# Autodesk Inventor assembly: !drivetrain
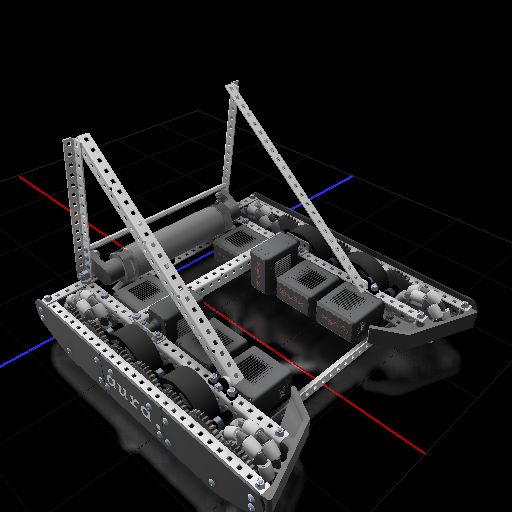
[picture p0: Inventor's stored thumbnail of the model, 512x512]
Saved by Autodesk Inventor 2025.2 (Build 292293000, 293)
## iProperties
Created: 2025-11-15
Part Number: !drivetrain
Document SubType Name: Assembly
Designer: cloudy
Author: cloudy
## Documents named in this file (53)
- C:\Users\cloudy\Documents\AURA_CAD\15\Drivetrain\!drivetrain.iam
- C:\Users\cloudy\Documents\AURA_CAD\15\Drivetrain\Wheels\Omni\2.75\2.75 Omni Assembly.iam
- C:\Users\cloudy\Documents\AURA_CAD\!lib\Structure\C Channel\Aluminum 1x2x1\Alu C 1x2x1x28.ipt
- C:\Users\cloudy\Documents\AURA_CAD\!lib\Structure\Hardware\Screw Steel - Star\SScrew Star Smooth 2.000.ipt
- C:\Users\cloudy\Documents\AURA_CAD\!lib\Structure\Hardware\Screw Steel - Star.ipt
- C:\Users\cloudy\Documents\AURA_CAD\!lib\Structure\Hardware\Nut Keps.ipt
- C:\Users\cloudy\Documents\AURA_CAD\!lib\Motion\Shaft LS\LS Pillow Bearing Block.ipt
- C:\Users\cloudy\Documents\AURA_CAD\!lib\Structure\C Channel\Aluminum 1x3x1 Half\Alu C Half 1x3x1x19.ipt
- C:\Users\cloudy\Documents\AURA_CAD\!lib\Structure\C Channel\Aluminum 1x2x1\Alu C 1x2x1x26.ipt
- C:\Users\cloudy\Documents\AURA_CAD\!lib\Structure\C Channel\Aluminum 1x3x1\Alu C 1x3x1x27.ipt
- C:\Users\cloudy\Documents\AURA_CAD\15\Drivetrain\Gears\26t_no_screwholes.ipt
- C:\Users\cloudy\Documents\AURA_CAD\!lib\Electronics\Motors with Screws\AluM-StarS.iam
- C:\Users\cloudy\Documents\AURA_CAD\!lib\Electronics\Motors with Screws.iam
- C:\Users\cloudy\Documents\AURA_CAD\15\Drivetrain\bearing_2 long.ipt
- C:\Users\cloudy\Documents\AURA_CAD\!lib\Motion\Spacers\Spacer Nylon .500 OD\NSpacer White .500 OD x .125.ipt
- C:\Users\cloudy\Documents\AURA_CAD\!lib\Motion\Spacers\Spacer Nylon .500 OD.ipt
- C:\Users\cloudy\Documents\AURA_CAD\!lib\Motion\Spacers\Spacer Nylon .375 OD\NSpacer .375 OD x .500.ipt
- C:\Users\cloudy\Documents\AURA_CAD\!lib\Motion\Spacers\Spacer Nylon .375 OD.ipt
- C:\Users\cloudy\Documents\AURA_CAD\!lib\Motion\Spacers\Spacer Nylon .375 OD\NSpacer .375 OD x .250.ipt
- C:\Users\cloudy\Documents\AURA_CAD\!lib\Motion\Shaft LS\Bearing Flat - Drilled.ipt
- C:\Users\cloudy\Documents\AURA_CAD\!lib\Motion\Shaft LS\Shaft Collar Metal\Shaft Collar No Screw.iam
- C:\Users\cloudy\Documents\AURA_CAD\!lib\Motion\Shaft LS\Shaft Collar Metal.iam
- C:\Users\cloudy\Documents\AURA_CAD\!lib\Structure\Standoff\Standoff 3.00.ipt
- C:\Users\cloudy\Documents\AURA_CAD\!lib\Structure\Standoff.ipt
- C:\Users\cloudy\Documents\AURA_CAD\!lib\Motion\Spacers\Spacer Nylon .375 OD\NSpacer .375 OD x .375.ipt
- C:\Users\cloudy\Documents\AURA_CAD\!lib\Motion\Spacers\Washer Steel\SWasher .375 OD x .062500.ipt
- C:\Users\cloudy\Documents\AURA_CAD\!lib\Motion\Spacers\Washer Steel.ipt
- C:\Users\cloudy\Documents\AURA_CAD\!lib\Structure\C Channel\Aluminum 1x3x1 Half\Alu C Half 1x3x1x3.ipt
- C:\Users\cloudy\Documents\AURA_CAD\!lib\Structure\C Channel\Aluminum 1x3x1 Half\Alu C Half 1x3x1x23.ipt
- C:\Users\cloudy\Documents\AURA_CAD\!lib\Structure\C Channel\Aluminum 1x3x1 Half\Alu C Half 1x3x1x15.ipt
- C:\Users\cloudy\Documents\AURA_CAD\!lib\Motion\Pneumatics\Legacy - SMC Pneumatics\Reservoir.ipt
- C:\Users\cloudy\Documents\AURA_CAD\15\cut_halfc.ipt
- C:\Users\cloudy\Documents\AURA_CAD\15\Drivetrain\Wheels\Traction\traction.iam
- C:\Users\cloudy\Documents\AURA_CAD\!lib\Structure\Hardware\Nut Nylock.ipt
- C:\Users\cloudy\Documents\AURA_CAD\15\ziptie.ipt
- C:\Users\cloudy\Documents\AURA_CAD\!lib\Motion\Shaft LS\Shaft LS Capped\Shaft LS Capped 3.0.ipt
- C:\Users\cloudy\Documents\AURA_CAD\!lib\Motion\Shaft LS\Shaft LS Capped.ipt
- C:\Users\cloudy\Documents\AURA_CAD\!lib\Structure\Hardware\Screw Steel - Star\SScrew Star Smooth .625.ipt
- C:\Users\cloudy\Documents\AURA_CAD\!lib\Structure\Hardware\Screw Steel - Star\SScrew Star Smooth .750.ipt
- C:\Users\cloudy\Documents\AURA_CAD\!lib\Structure\Hardware\Screw Steel - Star\SScrew Star Smooth .375.ipt
- C:\Users\cloudy\Documents\AURA_CAD\!lib\Structure\Hardware\Screw Steel - Star\SScrew Star Threaded 1.750.ipt
- C:\Users\cloudy\Documents\AURA_CAD\!lib\Structure\Hardware\Screw Steel - Star\SScrew Star Threaded .500.ipt
- C:\Users\cloudy\Documents\AURA_CAD\!lib\Structure\Standoff\Standoff 4.00.ipt
- C:\Users\cloudy\Documents\AURA_CAD\!lib\Structure\Standoff\Standoff .50.ipt
- C:\Users\cloudy\Documents\AURA_CAD\15\thing.ipt
- C:\Users\cloudy\Documents\AURA_CAD\15\thing_MIR.ipt
- C:\Users\cloudy\Documents\AURA_CAD\15\Drivetrain\funnel.ipt
- C:\Users\cloudy\Documents\AURA_CAD\!lib\Structure\C Channel\Aluminum 1x3x1 Half Thick Cut\Alu C Half Thick 1x3x1x20.ipt
- C:\Users\cloudy\Documents\AURA_CAD\!lib\Motion\Spacers\Spacer Nylon .375 OD\NSpacer .375 OD x .125.ipt
- C:\Users\cloudy\Documents\AURA_CAD\15\funnelFront.ipt
- C:\Users\cloudy\Documents\AURA_CAD\15\plate.ipt
- C:\Users\cloudy\Documents\AURA_CAD\!lib\Structure\Hardware\Screw Steel - Star\SScrew Star Smooth 1.250.ipt
- C:\Users\cloudy\Documents\AURA_CAD\!lib\Miscellaneous\iw_metal_02.bmp
## Components (277 placed, 43 different names)
1. Alu C 1x2x1x26:1 — Insert:10, Insert:19, Insert:20, Insert:26, Insert:36, Insert:40, Mate:22, Mate:23, Insert:41, Insert:42, Insert:43, Insert:47, Mate:24, Insert:51, Insert:67, Insert:90, Mate:37, Mate:38, Insert:102, Mate:44, Insert:110, Insert:117, Insert:122, Insert:123, Insert:126, Insert:144, Insert:154, Insert:157, Insert:163, Insert:164, Insert:165, Insert:170, Insert:171, Mate:92, Insert:313, Insert:315
2. SScrew Star Smooth 2.000:1 — Insert:10, Mate:26
3. 2.75 Omni Assembly:5 [sub-assembly] — Insert:46
4. SScrew Star Smooth 2.000:2 — Insert:20
5. SScrew Star Smooth 2.000:3 — Insert:19
6. 2.75 Omni Assembly:7 [sub-assembly] — Insert:44
7. Alu C Half 1x3x1x19:1 — Insert:26, Insert:161, Insert:162, Insert:264, Insert:265
8. Alu C 1x3x1x27:1 — Mate:15, Mate:16, Insert:32, Mate:34, Insert:72, Insert:108, Insert:126, Insert:141, Insert:150, Insert:155, Insert:156, Insert:158, Insert:167, Insert:168, Insert:169, Insert:257, Insert:258, Insert:260, Insert:262
9. 26t_no_screwholes:1 — Insert:52, Insert:56
10. 26t_no_screwholes:2 — Insert:53, Insert:55
11. 26t_no_screwholes:3 — Insert:54, Insert:57
12. Alu C 1x2x1x28:3 — Insert:32, Mate:26, Insert:52, Insert:53, Insert:54, Insert:58, Insert:59, Insert:60, Mate:27, Mate:28, Mate:29, Insert:61, Mate:30, Insert:62, Insert:63, Insert:64, Mate:31, Mate:32, Mate:33, Insert:124, Insert:125, Insert:127, Insert:128, Insert:129, Insert:130, Insert:131, Insert:132, Insert:133, Insert:134, Mate:49, Mate:50, Mate:51, Mate:52, Mate:53, Mate:54, Mate:55, Mate:56, Mate:57, Mate:58, Insert:135, Insert:136, Insert:137, Insert:138, Insert:152, Insert:283, Insert:284, Mate:93, Insert:294, Mate:95, Insert:297, Mate:97, Insert:314, Insert:316
13. AluM-StarS:1 [sub-assembly] — Insert:36, Mate:22
14. AluM-StarS:2 [sub-assembly] — Insert:40, Mate:23
15. AluM-StarS:3 [sub-assembly] — Insert:47, Mate:24
16. Nut Keps:1 — Insert:41, Insert:44
17. Nut Keps:2 — Insert:42, Insert:111
18. Nut Keps:3 — Insert:43, Insert:46
19. NSpacer White .500 OD x .125:2 — Insert:51
20. NSpacer .375 OD x .250:2 — Insert:56
21. NSpacer .375 OD x .250:3 — Insert:55
22. NSpacer .375 OD x .250:4 — Insert:57
23. bearing_2 long:3 — Insert:59, Mate:28
24. bearing_2 long:4 — Insert:61, Mate:30, Insert:112
25. bearing_2 long:5 — Insert:58, Mate:29
26. bearing_2 long:6 — Insert:60, Mate:27
27. Bearing Flat - Drilled:1 — Insert:62, Mate:33
28. Bearing Flat - Drilled:2 — Insert:64, Mate:31
29. Bearing Flat - Drilled:3 — Insert:63, Mate:32
30. Shaft Collar No Screw:1 [sub-assembly] — Insert:67, Mate:35, Insert:69, Insert:166
31. Shaft Collar No Screw:2 [sub-assembly] — Mate:34, Mate:35, Insert:68, Insert:74
32. Standoff 3.00:1 — Insert:70
33. NSpacer .375 OD x .500:5 — Insert:68
34. NSpacer .375 OD x .375:6 — Insert:69, Insert:70
35. NSpacer .375 OD x .500:7 — Insert:71, Insert:73
36. NSpacer .375 OD x .500:8 — Insert:71, Insert:72
37. SWasher .375 OD x .062500:1 — Insert:73
38. SWasher .375 OD x .062500:2 — Insert:74
39. Alu C Half 1x3x1x3:1 — Insert:90, Mate:37, Insert:91, Insert:147, Insert:148
40. AluM-StarS:7 [sub-assembly] — Insert:91, Mate:38
41. Alu C Half 1x3x1x23:1 — Mate:48, Insert:139, Insert:142
42. LS Pillow Bearing Block:2 — Insert:102, Mate:44, Insert:143, Insert:145, Insert:146
43. Shaft Collar No Screw:5 [sub-assembly] — Insert:108, Insert:109, Insert:159
44. Alu C Half 1x3x1x15:1 — Insert:109, Mate:48, Insert:160, Insert:270, Insert:279, Mate:90, Insert:280, Insert:281
45. Reservoir:1 — Mate:87, Mate:89
46. cut_halfc:1 — Insert:110, Insert:140, Insert:149, Mate:85
47. traction:1 [sub-assembly] — Insert:113
48. traction:2 [sub-assembly] — Insert:111, Insert:114
49. NSpacer .375 OD x .250:9 — Insert:112, Insert:113
50. Nut Nylock:1 — Insert:114
51. NSpacer .375 OD x .500:10 — Insert:116, Insert:117
52. NSpacer .375 OD x .375:11 — Insert:115
53. Shaft Collar No Screw:6 [sub-assembly] — Insert:115, Insert:116
54. NSpacer .375 OD x .500:12 — Insert:122
55. NSpacer .375 OD x .375:13
56. Shaft Collar No Screw:7 [sub-assembly]
57. NSpacer .375 OD x .500:14 — Insert:123
58. NSpacer .375 OD x .375:15
59. Shaft Collar No Screw:8 [sub-assembly]
60. ziptie:1 — Insert:125, Mate:56
61. ziptie:2 — Insert:127, Mate:57
62. ziptie:3 — Insert:128, Mate:55
63. ziptie:4 — Insert:124, Mate:58
64. ziptie:5 — Insert:129, Mate:53
65. ziptie:6 — Insert:130, Mate:54
66. ziptie:7 — Insert:131, Mate:52
67. ziptie:8 — Insert:133, Mate:50
68. ziptie:9 — Insert:132, Mate:51
69. ziptie:10 — Insert:134, Mate:49
70. Shaft LS Capped 3.0:1 — Insert:135
71. Shaft LS Capped 3.0:2 — Insert:136
72. Shaft LS Capped 3.0:3 — Insert:137
73. Shaft LS Capped 3.0:4 — Insert:138
74. NSpacer White .500 OD x .125:3 — Insert:139
75. NSpacer White .500 OD x .125:4 — Insert:140
76. NSpacer White .500 OD x .125:5 — Insert:141
77. SScrew Star Smooth .625:4 — Insert:142
78. Nut Nylock:2 — Insert:143
79. Nut Keps:4 — Insert:144
80. Nut Nylock:3 — Insert:146
81. Nut Nylock:4 — Insert:145
82. Nut Keps:5 — Insert:147
83. Nut Keps:6 — Insert:148
84. Nut Keps:7 — Insert:149
85. Nut Nylock:5 — Insert:150
86. NSpacer .375 OD x .500:16 — Insert:151, Insert:152
87. NSpacer .375 OD x .375:17 — Insert:151
88. NSpacer .375 OD x .500:18 — Insert:154
89. NSpacer .375 OD x .375:19
90. NSpacer .375 OD x .375:20 — Insert:155
91. NSpacer .375 OD x .375:21 — Insert:156
92. Nut Keps:8 — Insert:157
93. Nut Keps:9 — Insert:158
94. Nut Keps:10 — Insert:159
95. SScrew Star Smooth .625:5 — Insert:160
96. NSpacer .375 OD x .500:22 — Insert:161
97. SScrew Star Smooth .750:6 — Insert:162
98. SScrew Star Threaded .500:7 — Insert:164
99. SScrew Star Smooth .375:8 — Insert:163
100. SScrew Star Smooth .375:10 — Insert:165
101. SScrew Star Threaded .500:11 — Insert:166
102. SScrew Star Threaded 1.750:12 — Insert:167
103. SScrew Star Threaded 1.750:13 — Insert:168
104. SScrew Star Threaded 1.750:14 — Insert:169
105. SScrew Star Threaded .500:15 — Insert:170
106. SScrew Star Threaded .500:16 — Insert:171
107. Alu C 1x2x1x26:2 — Insert:172, Insert:173, Insert:174, Mate:60, Insert:178, Mate:61, Insert:179, Mate:62, Insert:180, Insert:182, Insert:183, Insert:185, Insert:186, Insert:197, Mate:71, Insert:204, Mate:72, Mate:73, Insert:206, Insert:213, Insert:216, Insert:219, Insert:239, Insert:246, Insert:248, Insert:252, Insert:253, Insert:255, Insert:256, Insert:258, Insert:263, Mate:91, Insert:317, Insert:319
108. SScrew Star Smooth 2.000:17 — Insert:172, Mate:59
109. 2.75 Omni Assembly:8 [sub-assembly] — Insert:184
110. SScrew Star Smooth 2.000:18 — Insert:173
111. SScrew Star Smooth 2.000:19 — Insert:174
112. 2.75 Omni Assembly:9 [sub-assembly] — Insert:181
113. 26t_no_screwholes:4 — Insert:177, Insert:187
114. 26t_no_screwholes:5 — Insert:176, Insert:188
115. 26t_no_screwholes:6 — Insert:175, Insert:189
116. Alu C 1x2x1x28:4 — Insert:175, Insert:176, Insert:177, Mate:59, Mate:63, Insert:190, Mate:64, Insert:191, Mate:65, Insert:192, Mate:66, Insert:193, Mate:67, Insert:194, Mate:68, Insert:195, Mate:69, Insert:196, Mate:75, Insert:222, Mate:76, Insert:223, Mate:77, Insert:224, Mate:78, Insert:225, Mate:79, Insert:226, Mate:80, Insert:227, Mate:81, Insert:228, Mate:82, Insert:229, Mate:83, Insert:230, Mate:84, Insert:231, Insert:232, Insert:233, Insert:234, Insert:235, Insert:244, Insert:257, Insert:282, Insert:285, Mate:94, Insert:295, Insert:296, Mate:96, Mate:98, Insert:318, Insert:320
117. AluM-StarS:8 [sub-assembly] — Mate:60, Insert:178
118. AluM-StarS:9 [sub-assembly] — Mate:61, Insert:179
119. AluM-StarS:10 [sub-assembly] — Mate:62, Insert:180
120. Nut Keps:11 — Insert:181, Insert:182
121. Nut Keps:12 — Insert:183, Insert:209
122. Nut Keps:13 — Insert:184, Insert:185
123. NSpacer White .500 OD x .125:6 — Insert:186
124. NSpacer .375 OD x .250:23 — Insert:187
125. NSpacer .375 OD x .250:24 — Insert:188
126. NSpacer .375 OD x .250:25 — Insert:189
127. bearing_2 long:7 — Mate:63, Insert:190
128. bearing_2 long:8 — Mate:64, Insert:191, Insert:211
129. bearing_2 long:9 — Mate:65, Insert:192
130. bearing_2 long:10 — Mate:66, Insert:193
131. Bearing Flat - Drilled:4 — Mate:67, Insert:194
132. Bearing Flat - Drilled:5 — Mate:68, Insert:195
133. Bearing Flat - Drilled:6 — Mate:69, Insert:196
134. Shaft Collar No Screw:9 [sub-assembly] — Insert:197, Mate:70, Insert:200, Insert:266
135. Shaft Collar No Screw:10 [sub-assembly] — Mate:70, Insert:198, Insert:203, Insert:261
136. Standoff 3.00:2 — Insert:199
137. NSpacer .375 OD x .500:26 — Insert:198
138. NSpacer .375 OD x .375:27 — Insert:199, Insert:200
139. NSpacer .375 OD x .500:28 — Insert:201, Insert:202
140. NSpacer .375 OD x .500:29 — Insert:201, Insert:262
141. SWasher .375 OD x .062500:3 — Insert:202, Insert:261
142. SWasher .375 OD x .062500:4 — Insert:203
143. Alu C Half 1x3x1x3:2 — Mate:71, Insert:204, Insert:205, Insert:242, Insert:243
144. AluM-StarS:11 [sub-assembly] — Mate:72, Insert:205
145. Alu C Half 1x3x1x23:2 — Insert:207, Mate:74, Insert:236, Insert:237
146. LS Pillow Bearing Block:3 — Mate:73, Insert:206, Insert:207, Insert:238, Insert:240, Insert:241
147. Shaft Collar No Screw:11 [sub-assembly] — Insert:208, Insert:249, Insert:259
148. Alu C Half 1x3x1x15:2 — Mate:74, Insert:208, Insert:250, Insert:269, Insert:271, Insert:272, Mate:88, Insert:273, Insert:274
149. traction:3 [sub-assembly] — Insert:210
150. traction:4 [sub-assembly] — Insert:209, Insert:212
151. NSpacer .375 OD x .250:30 — Insert:210, Insert:211
152. Nut Nylock:6 — Insert:212
153. NSpacer .375 OD x .500:31 — Insert:213, Insert:214
154. NSpacer .375 OD x .375:32 — Insert:215
155. Shaft Collar No Screw:12 [sub-assembly] — Insert:214, Insert:215
156. NSpacer .375 OD x .500:33 — Insert:216, Insert:217
157. NSpacer .375 OD x .375:34 — Insert:218
158. Shaft Collar No Screw:13 [sub-assembly] — Insert:217, Insert:218
159. NSpacer .375 OD x .500:35 — Insert:219, Insert:220
160. NSpacer .375 OD x .375:36 — Insert:221
161. Shaft Collar No Screw:14 [sub-assembly] — Insert:220, Insert:221
162. ziptie:11 — Mate:75, Insert:222
163. ziptie:12 — Mate:76, Insert:223
164. ziptie:13 — Mate:77, Insert:224
165. ziptie:14 — Mate:78, Insert:225
166. ziptie:15 — Mate:79, Insert:226
167. ziptie:16 — Mate:80, Insert:227
168. ziptie:17 — Mate:81, Insert:228
169. ziptie:18 — Mate:82, Insert:229
170. ziptie:19 — Mate:83, Insert:230
171. ziptie:20 — Mate:84, Insert:231
172. Shaft LS Capped 3.0:5 — Insert:232
173. Shaft LS Capped 3.0:6 — Insert:233
174. Shaft LS Capped 3.0:7 — Insert:234
175. Shaft LS Capped 3.0:8 — Insert:235
176. NSpacer White .500 OD x .125:7 — Insert:236
177. NSpacer White .500 OD x .125:8 — Mate:85
178. NSpacer White .500 OD x .125:9 — Insert:259, Insert:260
179. SScrew Star Smooth .625:20 — Insert:237
180. Nut Nylock:7 — Insert:238
181. Nut Keps:14 — Insert:239, Mate:86
182. Nut Nylock:8 — Insert:240
183. Nut Nylock:9 — Insert:241
184. Nut Keps:15 — Insert:242
185. Nut Keps:16 — Insert:243
186. Nut Keps:17
187. Nut Nylock:10
188. NSpacer .375 OD x .500:37 — Insert:244, Insert:245
189. NSpacer .375 OD x .375:38 — Insert:245
190. NSpacer .375 OD x .500:39 — Insert:246, Insert:247
191. NSpacer .375 OD x .375:40 — Insert:247
192. NSpacer .375 OD x .375:41
193. NSpacer .375 OD x .375:42
194. Nut Keps:18 — Insert:248
195. Nut Keps:19
196. Nut Keps:20 — Insert:249
197. SScrew Star Smooth .625:21 — Insert:250
198. NSpacer .375 OD x .500:43 — Insert:265, Mate:86
199. SScrew Star Smooth .750:22 — Insert:264
200. SScrew Star Smooth .375:24 — Insert:252
201. SScrew Star Smooth .375:25 — Insert:253
202. SScrew Star Threaded 1.750:27
203. SScrew Star Threaded 1.750:28
204. SScrew Star Threaded 1.750:29
205. SScrew Star Threaded .500:30 — Insert:255
206. SScrew Star Threaded .500:31 — Insert:256
207. SScrew Star Threaded .500:32 — Insert:263
208. SScrew Star Threaded .500:33 — Insert:266
209. Standoff 4.00:3 — Insert:267
210. Standoff 4.00:4 — Insert:268, Insert:269
211. Standoff .50:5 — Insert:267, Insert:268
212. SScrew Star Smooth .625:34 — Insert:271
213. SScrew Star Smooth .625:35 — Insert:270
214. thing:1 — Insert:272, Mate:88, Mate:89, Insert:275, Insert:276
215. SScrew Star Smooth .625:36 — Insert:274
216. SScrew Star Smooth .625:37 — Insert:273
217. Nut Nylock:11 — Insert:275
218. Nut Nylock:13 — Insert:276
219. thing_MIR:1 — Insert:277, Insert:278, Insert:279, Mate:90
220. SScrew Star Smooth .625:38 — Insert:281
221. SScrew Star Smooth .625:39 — Insert:280
222. Nut Nylock:14 — Insert:277
223. Nut Nylock:15 — Insert:278
224. funnel:2 — Insert:282, Mate:91
225. funnel:3 — Insert:283, Mate:92
226. Alu C Half Thick 1x3x1x20:1 — Insert:284, Mate:93, Insert:287, Insert:289, Flush:1
227. Alu C Half Thick 1x3x1x20:2 — Insert:285, Mate:94, Insert:291, Insert:293, Insert:298
228. NSpacer .375 OD x .500:44 — Insert:286, Insert:287
229. NSpacer .375 OD x .125:45 — Insert:286
230. NSpacer .375 OD x .500:46 — Insert:289
231. NSpacer .375 OD x .125:47
232. NSpacer .375 OD x .500:48 — Insert:291
233. NSpacer .375 OD x .125:49
234. NSpacer .375 OD x .500:50 — Insert:293
235. NSpacer .375 OD x .125:51
236. funnelFront:1 — Insert:295, Insert:321, Insert:322, Insert:323, Insert:324, Insert:325
237. funnelFront:2 — Insert:294, Mate:95, Insert:299, Insert:300, Insert:301, Insert:302, Insert:303
238. funnelFront:3 — Insert:296, Mate:96, Insert:330, Insert:331, Insert:332, Insert:333, Insert:334
239. funnelFront:4 — Insert:297, Mate:97, Insert:308, Insert:309, Insert:310, Insert:311, Insert:312
240. plate:1 — Flush:1, Insert:304, Insert:305, Insert:306, Insert:307
241. plate:2 — Insert:298, Mate:98, Insert:326, Insert:327, Insert:328, Insert:329
242. SScrew Star Smooth .375:40 — Insert:301
243. SScrew Star Smooth .375:41 — Insert:302
244. SScrew Star Smooth .375:42 — Insert:300
245. SScrew Star Smooth .375:43 — Insert:303
246. SScrew Star Smooth .375:44 — Insert:299
247. SScrew Star Smooth .375:45 — Insert:310
248. SScrew Star Smooth .375:46 — Insert:311
249. SScrew Star Smooth .375:47 — Insert:309
250. SScrew Star Smooth .375:48 — Insert:312
251. SScrew Star Smooth .375:49 — Insert:307
252. SScrew Star Smooth .375:50 — Insert:308
253. SScrew Star Smooth .375:51 — Insert:306
254. SScrew Star Smooth .375:52 — Insert:304
255. SScrew Star Smooth .375:53 — Insert:305
256. Nut Nylock:16 — Insert:315
257. SScrew Star Smooth 1.250:54 — Insert:314
258. Nut Nylock:17 — Insert:316
259. SScrew Star Smooth 1.250:55 — Insert:313
260. Nut Nylock:18 — Insert:319
261. SScrew Star Smooth 1.250:56 — Insert:318
262. Nut Nylock:19 — Insert:320
263. SScrew Star Smooth 1.250:57 — Insert:317
264. SScrew Star Smooth .375:58 — Insert:321
265. SScrew Star Smooth .375:59 — Insert:325
266. SScrew Star Smooth .375:60 — Insert:322
267. SScrew Star Smooth .375:61 — Insert:324
268. SScrew Star Smooth .375:62 — Insert:323
269. SScrew Star Smooth .375:63 — Insert:333
270. SScrew Star Smooth .375:64 — Insert:329
271. SScrew Star Smooth .375:65 — Insert:330
272. SScrew Star Smooth .375:66 — Insert:328
273. SScrew Star Smooth .375:67 — Insert:334
274. SScrew Star Smooth .375:68 — Insert:332
275. SScrew Star Smooth .375:69 — Insert:331
276. SScrew Star Smooth .375:70 — Insert:326
277. SScrew Star Smooth .375:71 — Insert:327
## Relationships (334: Insert 264, Mate 69, Flush 1)
- Insert:10: Alu C 1x2x1x26:1 ↔ SScrew Star Smooth 2.000:1
- Insert:19: Alu C 1x2x1x26:1 ↔ SScrew Star Smooth 2.000:3
- Insert:20: Alu C 1x2x1x26:1 ↔ SScrew Star Smooth 2.000:2
- Insert:26 (12.7 mm): Alu C 1x2x1x26:1 ↔ Alu C Half 1x3x1x19:1
- Mate:15: Alu C 1x3x1x27:1
- Mate:16: Alu C 1x3x1x27:1
- Insert:32: Alu C 1x3x1x27:1 ↔ Alu C 1x2x1x28:3
- Insert:36: Alu C 1x2x1x26:1 ↔ AluM-StarS:1
- Insert:40: Alu C 1x2x1x26:1 ↔ AluM-StarS:2
- Mate:22: Alu C 1x2x1x26:1 ↔ AluM-StarS:1
- Mate:23: Alu C 1x2x1x26:1 ↔ AluM-StarS:2
- Insert:41: Alu C 1x2x1x26:1 ↔ Nut Keps:1
- Insert:42: Alu C 1x2x1x26:1 ↔ Nut Keps:2
- Insert:43: Alu C 1x2x1x26:1 ↔ Nut Keps:3
- Insert:44 (0.7937 mm): 2.75 Omni Assembly:7 ↔ Nut Keps:1
- Insert:46 (0.7937 mm): 2.75 Omni Assembly:5 ↔ Nut Keps:3
- Insert:47: Alu C 1x2x1x26:1 ↔ AluM-StarS:3
- Mate:24: Alu C 1x2x1x26:1 ↔ AluM-StarS:3
- Insert:51: Alu C 1x2x1x26:1 ↔ NSpacer White .500 OD x .125:2
- Mate:26: SScrew Star Smooth 2.000:1 ↔ Alu C 1x2x1x28:3
- Insert:52 (13.4938 mm): 26t_no_screwholes:1 ↔ Alu C 1x2x1x28:3
- Insert:53 (13.4938 mm): 26t_no_screwholes:2 ↔ Alu C 1x2x1x28:3
- Insert:54 (13.4938 mm): 26t_no_screwholes:3 ↔ Alu C 1x2x1x28:3
- Insert:55: 26t_no_screwholes:2 ↔ NSpacer .375 OD x .250:3
- Insert:56: 26t_no_screwholes:1 ↔ NSpacer .375 OD x .250:2
- Insert:57: 26t_no_screwholes:3 ↔ NSpacer .375 OD x .250:4
- Insert:58: Alu C 1x2x1x28:3 ↔ bearing_2 long:5
- Insert:59: Alu C 1x2x1x28:3 ↔ bearing_2 long:3
- Insert:60: Alu C 1x2x1x28:3 ↔ bearing_2 long:6
- Mate:27: Alu C 1x2x1x28:3 ↔ bearing_2 long:6
- Mate:28: Alu C 1x2x1x28:3 ↔ bearing_2 long:3
- Mate:29: Alu C 1x2x1x28:3 ↔ bearing_2 long:5
- Insert:61: Alu C 1x2x1x28:3 ↔ bearing_2 long:4
- Mate:30: Alu C 1x2x1x28:3 ↔ bearing_2 long:4
- Insert:62: Alu C 1x2x1x28:3 ↔ Bearing Flat - Drilled:1
- Insert:63: Alu C 1x2x1x28:3 ↔ Bearing Flat - Drilled:3
- Insert:64: Alu C 1x2x1x28:3 ↔ Bearing Flat - Drilled:2
- Mate:31: Alu C 1x2x1x28:3 ↔ Bearing Flat - Drilled:2
- Mate:32: Alu C 1x2x1x28:3 ↔ Bearing Flat - Drilled:3
- Mate:33: Alu C 1x2x1x28:3 ↔ Bearing Flat - Drilled:1
- Insert:67: Alu C 1x2x1x26:1 ↔ Shaft Collar No Screw:1
- Mate:34: Alu C 1x3x1x27:1 ↔ Shaft Collar No Screw:2
- Mate:35: Shaft Collar No Screw:1 ↔ Shaft Collar No Screw:2
- Insert:68: Shaft Collar No Screw:2 ↔ NSpacer .375 OD x .500:5
- Insert:69: Shaft Collar No Screw:1 ↔ NSpacer .375 OD x .375:6
- Insert:70: Standoff 3.00:1 ↔ NSpacer .375 OD x .375:6
- Insert:71: NSpacer .375 OD x .500:7 ↔ NSpacer .375 OD x .500:8
- Insert:72: Alu C 1x3x1x27:1 ↔ NSpacer .375 OD x .500:8
- Insert:73: NSpacer .375 OD x .500:7 ↔ SWasher .375 OD x .062500:1
- Insert:74: Shaft Collar No Screw:2 ↔ SWasher .375 OD x .062500:2
- Insert:90: Alu C 1x2x1x26:1 ↔ Alu C Half 1x3x1x3:1
- Mate:37: Alu C 1x2x1x26:1 ↔ Alu C Half 1x3x1x3:1
- Insert:91: Alu C Half 1x3x1x3:1 ↔ AluM-StarS:7
- Mate:38: Alu C 1x2x1x26:1 ↔ AluM-StarS:7
- [Insert] (3.175 mm): Alu C Half 1x3x1x23:1 ↔ LS Pillow Bearing Block:2
- Insert:102: Alu C 1x2x1x26:1 ↔ LS Pillow Bearing Block:2
- Mate:44: Alu C 1x2x1x26:1 ↔ LS Pillow Bearing Block:2
- Insert:108 (3.175 mm): Alu C 1x3x1x27:1 ↔ Shaft Collar No Screw:5
- Insert:109 (1.5875 mm): Shaft Collar No Screw:5 ↔ Alu C Half 1x3x1x15:1
- Mate:48: Alu C Half 1x3x1x23:1 ↔ Alu C Half 1x3x1x15:1
- Insert:110 (4.7625 mm): Alu C 1x2x1x26:1 ↔ cut_halfc:1
- Insert:111: Nut Keps:2 ↔ traction:2
- Insert:112 (0.7937 mm): bearing_2 long:4 ↔ NSpacer .375 OD x .250:9
- Insert:113: traction:1 ↔ NSpacer .375 OD x .250:9
- Insert:114: traction:2 ↔ Nut Nylock:1
- Insert:115: NSpacer .375 OD x .375:11 ↔ Shaft Collar No Screw:6
- Insert:116: NSpacer .375 OD x .500:10 ↔ Shaft Collar No Screw:6
- Insert:117 (1.016 mm): Alu C 1x2x1x26:1 ↔ NSpacer .375 OD x .500:10
- [Insert]: NSpacer .375 OD x .375:13 ↔ Shaft Collar No Screw:7
- [Insert]: NSpacer .375 OD x .500:12 ↔ Shaft Collar No Screw:7
- [Insert]: NSpacer .375 OD x .375:15 ↔ Shaft Collar No Screw:8
- [Insert]: NSpacer .375 OD x .500:14 ↔ Shaft Collar No Screw:8
- Insert:122 (1.016 mm): Alu C 1x2x1x26:1 ↔ NSpacer .375 OD x .500:12
- Insert:123 (1.016 mm): Alu C 1x2x1x26:1 ↔ NSpacer .375 OD x .500:14
- Insert:124: Alu C 1x2x1x28:3 ↔ ziptie:4
- Insert:125: Alu C 1x2x1x28:3 ↔ ziptie:1
- Insert:126: Alu C 1x2x1x26:1 ↔ Alu C 1x3x1x27:1
- Insert:127: Alu C 1x2x1x28:3 ↔ ziptie:2
- Insert:128: Alu C 1x2x1x28:3 ↔ ziptie:3
- Insert:129: Alu C 1x2x1x28:3 ↔ ziptie:5
- Insert:130: Alu C 1x2x1x28:3 ↔ ziptie:6
- Insert:131: Alu C 1x2x1x28:3 ↔ ziptie:7
- Insert:132: Alu C 1x2x1x28:3 ↔ ziptie:9
- Insert:133: Alu C 1x2x1x28:3 ↔ ziptie:8
- Insert:134: Alu C 1x2x1x28:3 ↔ ziptie:10
- Mate:49: Alu C 1x2x1x28:3 ↔ ziptie:10
- Mate:50: Alu C 1x2x1x28:3 ↔ ziptie:8
- Mate:51: Alu C 1x2x1x28:3 ↔ ziptie:9
- Mate:52: Alu C 1x2x1x28:3 ↔ ziptie:7
- Mate:53: Alu C 1x2x1x28:3 ↔ ziptie:5
- Mate:54: Alu C 1x2x1x28:3 ↔ ziptie:6
- Mate:55: Alu C 1x2x1x28:3 ↔ ziptie:3
- Mate:56: Alu C 1x2x1x28:3 ↔ ziptie:1
- Mate:57: Alu C 1x2x1x28:3 ↔ ziptie:2
- Mate:58: Alu C 1x2x1x28:3 ↔ ziptie:4
- Insert:135: Alu C 1x2x1x28:3 ↔ Shaft LS Capped 3.0:1
- Insert:136: Alu C 1x2x1x28:3 ↔ Shaft LS Capped 3.0:2
- Insert:137: Alu C 1x2x1x28:3 ↔ Shaft LS Capped 3.0:3
- Insert:138: Alu C 1x2x1x28:3 ↔ Shaft LS Capped 3.0:4
- Insert:139: Alu C Half 1x3x1x23:1 ↔ NSpacer White .500 OD x .125:3
- Insert:140: cut_halfc:1 ↔ NSpacer White .500 OD x .125:4
- Insert:141: Alu C 1x3x1x27:1 ↔ NSpacer White .500 OD x .125:5
- Insert:142: Alu C Half 1x3x1x23:1 ↔ SScrew Star Smooth .625:4
- Insert:143: LS Pillow Bearing Block:2 ↔ Nut Nylock:2
- Insert:144: Alu C 1x2x1x26:1 ↔ Nut Keps:4
- Insert:145: LS Pillow Bearing Block:2 ↔ Nut Nylock:4
- Insert:146: LS Pillow Bearing Block:2 ↔ Nut Nylock:3
- Insert:147: Alu C Half 1x3x1x3:1 ↔ Nut Keps:5
- Insert:148: Alu C Half 1x3x1x3:1 ↔ Nut Keps:6
- Insert:149: cut_halfc:1 ↔ Nut Keps:7
- Insert:150: Alu C 1x3x1x27:1 ↔ Nut Nylock:5
- Insert:151: NSpacer .375 OD x .500:16 ↔ NSpacer .375 OD x .375:17
- Insert:152: Alu C 1x2x1x28:3 ↔ NSpacer .375 OD x .500:16
- [Insert]: NSpacer .375 OD x .500:18 ↔ NSpacer .375 OD x .375:19
- Insert:154: Alu C 1x2x1x26:1 ↔ NSpacer .375 OD x .500:18
- Insert:155: Alu C 1x3x1x27:1 ↔ NSpacer .375 OD x .375:20
- Insert:156: Alu C 1x3x1x27:1 ↔ NSpacer .375 OD x .375:21
- Insert:157: Alu C 1x2x1x26:1 ↔ Nut Keps:8
- Insert:158: Alu C 1x3x1x27:1 ↔ Nut Keps:9
- Insert:159: Shaft Collar No Screw:5 ↔ Nut Keps:10
- Insert:160: Alu C Half 1x3x1x15:1 ↔ SScrew Star Smooth .625:5
- Insert:161: Alu C Half 1x3x1x19:1 ↔ NSpacer .375 OD x .500:22
- Insert:162: Alu C Half 1x3x1x19:1 ↔ SScrew Star Smooth .750:6
- Insert:163: Alu C 1x2x1x26:1 ↔ SScrew Star Smooth .375:8
- Insert:164: Alu C 1x2x1x26:1 ↔ SScrew Star Threaded .500:7
- Insert:165: Alu C 1x2x1x26:1 ↔ SScrew Star Smooth .375:10
- Insert:166: Shaft Collar No Screw:1 ↔ SScrew Star Threaded .500:11
- Insert:167: Alu C 1x3x1x27:1 ↔ SScrew Star Threaded 1.750:12
- Insert:168: Alu C 1x3x1x27:1 ↔ SScrew Star Threaded 1.750:13
- Insert:169: Alu C 1x3x1x27:1 ↔ SScrew Star Threaded 1.750:14
- Insert:170: Alu C 1x2x1x26:1 ↔ SScrew Star Threaded .500:15
- Insert:171: Alu C 1x2x1x26:1 ↔ SScrew Star Threaded .500:16
- Insert:172: Alu C 1x2x1x26:2 ↔ SScrew Star Smooth 2.000:17
- Insert:173: Alu C 1x2x1x26:2 ↔ SScrew Star Smooth 2.000:18
- Insert:174: Alu C 1x2x1x26:2 ↔ SScrew Star Smooth 2.000:19
- Insert:175 (13.4938 mm): 26t_no_screwholes:6 ↔ Alu C 1x2x1x28:4
- Insert:176 (13.4938 mm): 26t_no_screwholes:5 ↔ Alu C 1x2x1x28:4
- Insert:177 (13.4938 mm): 26t_no_screwholes:4 ↔ Alu C 1x2x1x28:4
- Mate:59: SScrew Star Smooth 2.000:17 ↔ Alu C 1x2x1x28:4
- Mate:60: Alu C 1x2x1x26:2 ↔ AluM-StarS:8
- Insert:178: Alu C 1x2x1x26:2 ↔ AluM-StarS:8
- Mate:61: Alu C 1x2x1x26:2 ↔ AluM-StarS:9
- Insert:179: Alu C 1x2x1x26:2 ↔ AluM-StarS:9
- Mate:62: Alu C 1x2x1x26:2 ↔ AluM-StarS:10
- Insert:180: Alu C 1x2x1x26:2 ↔ AluM-StarS:10
- Insert:181 (0.7937 mm): 2.75 Omni Assembly:9 ↔ Nut Keps:11
- Insert:182: Alu C 1x2x1x26:2 ↔ Nut Keps:11
- Insert:183: Alu C 1x2x1x26:2 ↔ Nut Keps:12
- Insert:184 (0.7937 mm): 2.75 Omni Assembly:8 ↔ Nut Keps:13
- Insert:185: Alu C 1x2x1x26:2 ↔ Nut Keps:13
- Insert:186: Alu C 1x2x1x26:2 ↔ NSpacer White .500 OD x .125:6
- Insert:187: 26t_no_screwholes:4 ↔ NSpacer .375 OD x .250:23
- Insert:188: 26t_no_screwholes:5 ↔ NSpacer .375 OD x .250:24
- Insert:189: 26t_no_screwholes:6 ↔ NSpacer .375 OD x .250:25
- Mate:63: Alu C 1x2x1x28:4 ↔ bearing_2 long:7
- Insert:190: Alu C 1x2x1x28:4 ↔ bearing_2 long:7
- Mate:64: Alu C 1x2x1x28:4 ↔ bearing_2 long:8
- Insert:191: Alu C 1x2x1x28:4 ↔ bearing_2 long:8
- Mate:65: Alu C 1x2x1x28:4 ↔ bearing_2 long:9
- Insert:192: Alu C 1x2x1x28:4 ↔ bearing_2 long:9
- Mate:66: Alu C 1x2x1x28:4 ↔ bearing_2 long:10
- Insert:193: Alu C 1x2x1x28:4 ↔ bearing_2 long:10
- Mate:67: Alu C 1x2x1x28:4 ↔ Bearing Flat - Drilled:4
- Insert:194: Alu C 1x2x1x28:4 ↔ Bearing Flat - Drilled:4
- Mate:68: Alu C 1x2x1x28:4 ↔ Bearing Flat - Drilled:5
- Insert:195: Alu C 1x2x1x28:4 ↔ Bearing Flat - Drilled:5
- Mate:69: Alu C 1x2x1x28:4 ↔ Bearing Flat - Drilled:6
- Insert:196: Alu C 1x2x1x28:4 ↔ Bearing Flat - Drilled:6
- Insert:197: Alu C 1x2x1x26:2 ↔ Shaft Collar No Screw:9
- Mate:70: Shaft Collar No Screw:9 ↔ Shaft Collar No Screw:10
- Insert:198: Shaft Collar No Screw:10 ↔ NSpacer .375 OD x .500:26
- Insert:199: Standoff 3.00:2 ↔ NSpacer .375 OD x .375:27
- Insert:200: Shaft Collar No Screw:9 ↔ NSpacer .375 OD x .375:27
- Insert:201: NSpacer .375 OD x .500:28 ↔ NSpacer .375 OD x .500:29
- Insert:202: NSpacer .375 OD x .500:28 ↔ SWasher .375 OD x .062500:3
- Insert:203: Shaft Collar No Screw:10 ↔ SWasher .375 OD x .062500:4
- Mate:71: Alu C 1x2x1x26:2 ↔ Alu C Half 1x3x1x3:2
- Insert:204: Alu C 1x2x1x26:2 ↔ Alu C Half 1x3x1x3:2
- Mate:72: Alu C 1x2x1x26:2 ↔ AluM-StarS:11
- Insert:205: Alu C Half 1x3x1x3:2 ↔ AluM-StarS:11
- Mate:73: Alu C 1x2x1x26:2 ↔ LS Pillow Bearing Block:3
- Insert:206: Alu C 1x2x1x26:2 ↔ LS Pillow Bearing Block:3
- Insert:207 (3.175 mm): Alu C Half 1x3x1x23:2 ↔ LS Pillow Bearing Block:3
- Mate:74: Alu C Half 1x3x1x23:2 ↔ Alu C Half 1x3x1x15:2
- Insert:208 (1.5875 mm): Shaft Collar No Screw:11 ↔ Alu C Half 1x3x1x15:2
- Insert:209: Nut Keps:12 ↔ traction:4
- Insert:210: traction:3 ↔ NSpacer .375 OD x .250:30
- Insert:211 (0.7937 mm): bearing_2 long:8 ↔ NSpacer .375 OD x .250:30
- Insert:212: traction:4 ↔ Nut Nylock:6
- Insert:213 (1.016 mm): Alu C 1x2x1x26:2 ↔ NSpacer .375 OD x .500:31
- Insert:214: NSpacer .375 OD x .500:31 ↔ Shaft Collar No Screw:12
- Insert:215: NSpacer .375 OD x .375:32 ↔ Shaft Collar No Screw:12
- Insert:216 (1.016 mm): Alu C 1x2x1x26:2 ↔ NSpacer .375 OD x .500:33
- Insert:217: NSpacer .375 OD x .500:33 ↔ Shaft Collar No Screw:13
- Insert:218: NSpacer .375 OD x .375:34 ↔ Shaft Collar No Screw:13
- Insert:219 (1.016 mm): Alu C 1x2x1x26:2 ↔ NSpacer .375 OD x .500:35
- Insert:220: NSpacer .375 OD x .500:35 ↔ Shaft Collar No Screw:14
- Insert:221: NSpacer .375 OD x .375:36 ↔ Shaft Collar No Screw:14
- Mate:75: Alu C 1x2x1x28:4 ↔ ziptie:11
- Insert:222: Alu C 1x2x1x28:4 ↔ ziptie:11
- Mate:76: Alu C 1x2x1x28:4 ↔ ziptie:12
- Insert:223: Alu C 1x2x1x28:4 ↔ ziptie:12
- Mate:77: Alu C 1x2x1x28:4 ↔ ziptie:13
- Insert:224: Alu C 1x2x1x28:4 ↔ ziptie:13
- Mate:78: Alu C 1x2x1x28:4 ↔ ziptie:14
- Insert:225: Alu C 1x2x1x28:4 ↔ ziptie:14
- Mate:79: Alu C 1x2x1x28:4 ↔ ziptie:15
- Insert:226: Alu C 1x2x1x28:4 ↔ ziptie:15
- Mate:80: Alu C 1x2x1x28:4 ↔ ziptie:16
- Insert:227: Alu C 1x2x1x28:4 ↔ ziptie:16
- Mate:81: Alu C 1x2x1x28:4 ↔ ziptie:17
- Insert:228: Alu C 1x2x1x28:4 ↔ ziptie:17
- Mate:82: Alu C 1x2x1x28:4 ↔ ziptie:18
- Insert:229: Alu C 1x2x1x28:4 ↔ ziptie:18
- Mate:83: Alu C 1x2x1x28:4 ↔ ziptie:19
- Insert:230: Alu C 1x2x1x28:4 ↔ ziptie:19
- Mate:84: Alu C 1x2x1x28:4 ↔ ziptie:20
- Insert:231: Alu C 1x2x1x28:4 ↔ ziptie:20
- Insert:232: Alu C 1x2x1x28:4 ↔ Shaft LS Capped 3.0:5
- Insert:233: Alu C 1x2x1x28:4 ↔ Shaft LS Capped 3.0:6
- Insert:234: Alu C 1x2x1x28:4 ↔ Shaft LS Capped 3.0:7
- Insert:235: Alu C 1x2x1x28:4 ↔ Shaft LS Capped 3.0:8
- Insert:236: Alu C Half 1x3x1x23:2 ↔ NSpacer White .500 OD x .125:7
- Insert:237: Alu C Half 1x3x1x23:2 ↔ SScrew Star Smooth .625:20
- Insert:238: LS Pillow Bearing Block:3 ↔ Nut Nylock:7
- Insert:239: Alu C 1x2x1x26:2 ↔ Nut Keps:14
- Insert:240: LS Pillow Bearing Block:3 ↔ Nut Nylock:8
- Insert:241: LS Pillow Bearing Block:3 ↔ Nut Nylock:9
- Insert:242: Alu C Half 1x3x1x3:2 ↔ Nut Keps:15
- Insert:243: Alu C Half 1x3x1x3:2 ↔ Nut Keps:16
- Insert:244: Alu C 1x2x1x28:4 ↔ NSpacer .375 OD x .500:37
- Insert:245: NSpacer .375 OD x .500:37 ↔ NSpacer .375 OD x .375:38
- Insert:246: Alu C 1x2x1x26:2 ↔ NSpacer .375 OD x .500:39
- Insert:247: NSpacer .375 OD x .500:39 ↔ NSpacer .375 OD x .375:40
- Insert:248: Alu C 1x2x1x26:2 ↔ Nut Keps:18
- Insert:249: Shaft Collar No Screw:11 ↔ Nut Keps:20
- Insert:250: Alu C Half 1x3x1x15:2 ↔ SScrew Star Smooth .625:21
- Insert:252: Alu C 1x2x1x26:2 ↔ SScrew Star Smooth .375:24
- Insert:253: Alu C 1x2x1x26:2 ↔ SScrew Star Smooth .375:25
- Insert:255: Alu C 1x2x1x26:2 ↔ SScrew Star Threaded .500:30
- Insert:256: Alu C 1x2x1x26:2 ↔ SScrew Star Threaded .500:31
- Insert:257: Alu C 1x3x1x27:1 ↔ Alu C 1x2x1x28:4
- Insert:258: Alu C 1x3x1x27:1 ↔ Alu C 1x2x1x26:2
- Insert:259: Shaft Collar No Screw:11 ↔ NSpacer White .500 OD x .125:9
- Insert:260: Alu C 1x3x1x27:1 ↔ NSpacer White .500 OD x .125:9
- Insert:261: Shaft Collar No Screw:10 ↔ SWasher .375 OD x .062500:3
- Insert:262: Alu C 1x3x1x27:1 ↔ NSpacer .375 OD x .500:29
- Mate:85: cut_halfc:1 ↔ NSpacer White .500 OD x .125:8
- Insert:263: Alu C 1x2x1x26:2 ↔ SScrew Star Threaded .500:32
- Insert:264: Alu C Half 1x3x1x19:1 ↔ SScrew Star Smooth .750:22
- Insert:265: Alu C Half 1x3x1x19:1 ↔ NSpacer .375 OD x .500:43
- Mate:86: Nut Keps:14 ↔ NSpacer .375 OD x .500:43
- Insert:266: Shaft Collar No Screw:9 ↔ SScrew Star Threaded .500:33
- Insert:267: Standoff 4.00:3 ↔ Standoff .50:5
- Insert:268: Standoff 4.00:4 ↔ Standoff .50:5
- Insert:269: Alu C Half 1x3x1x15:2 ↔ Standoff 4.00:4
- Insert:270: Alu C Half 1x3x1x15:1 ↔ SScrew Star Smooth .625:35
- Insert:271: Alu C Half 1x3x1x15:2 ↔ SScrew Star Smooth .625:34
- Mate:87 (-100 mm): Reservoir:1
- Insert:272: Alu C Half 1x3x1x15:2 ↔ thing:1
- Mate:88: Alu C Half 1x3x1x15:2 ↔ thing:1
- Mate:89: Reservoir:1 ↔ thing:1
- Insert:273: Alu C Half 1x3x1x15:2 ↔ SScrew Star Smooth .625:37
- Insert:274: Alu C Half 1x3x1x15:2 ↔ SScrew Star Smooth .625:36
- Insert:275: thing:1 ↔ Nut Nylock:11
- Insert:276: thing:1 ↔ Nut Nylock:13
- Insert:277: thing_MIR:1 ↔ Nut Nylock:14
- Insert:278: thing_MIR:1 ↔ Nut Nylock:15
- Insert:279: Alu C Half 1x3x1x15:1 ↔ thing_MIR:1
- Mate:90: Alu C Half 1x3x1x15:1 ↔ thing_MIR:1
- Insert:280: Alu C Half 1x3x1x15:1 ↔ SScrew Star Smooth .625:39
- Insert:281: Alu C Half 1x3x1x15:1 ↔ SScrew Star Smooth .625:38
- Insert:282: Alu C 1x2x1x28:4 ↔ funnel:2
- Mate:91: Alu C 1x2x1x26:2 ↔ funnel:2
- Insert:283: Alu C 1x2x1x28:3 ↔ funnel:3
- Mate:92: Alu C 1x2x1x26:1 ↔ funnel:3
- Insert:284 (15.875 mm): Alu C 1x2x1x28:3 ↔ Alu C Half Thick 1x3x1x20:1
- Mate:93: Alu C 1x2x1x28:3 ↔ Alu C Half Thick 1x3x1x20:1
- Insert:285 (15.875 mm): Alu C 1x2x1x28:4 ↔ Alu C Half Thick 1x3x1x20:2
- Mate:94: Alu C 1x2x1x28:4 ↔ Alu C Half Thick 1x3x1x20:2
- Insert:286: NSpacer .375 OD x .500:44 ↔ NSpacer .375 OD x .125:45
- Insert:287: Alu C Half Thick 1x3x1x20:1 ↔ NSpacer .375 OD x .500:44
- [Insert]: NSpacer .375 OD x .500:46 ↔ NSpacer .375 OD x .125:47
- Insert:289: Alu C Half Thick 1x3x1x20:1 ↔ NSpacer .375 OD x .500:46
- [Insert]: NSpacer .375 OD x .500:48 ↔ NSpacer .375 OD x .125:49
- Insert:291: Alu C Half Thick 1x3x1x20:2 ↔ NSpacer .375 OD x .500:48
- [Insert]: NSpacer .375 OD x .500:50 ↔ NSpacer .375 OD x .125:51
- Insert:293: Alu C Half Thick 1x3x1x20:2 ↔ NSpacer .375 OD x .500:50
- Insert:294: Alu C 1x2x1x28:3 ↔ funnelFront:2
- Mate:95: Alu C 1x2x1x28:3 ↔ funnelFront:2
- Insert:295: Alu C 1x2x1x28:4 ↔ funnelFront:1
- Insert:296: Alu C 1x2x1x28:4 ↔ funnelFront:3
- Mate:96: Alu C 1x2x1x28:4 ↔ funnelFront:3
- Insert:297: Alu C 1x2x1x28:3 ↔ funnelFront:4
- Mate:97: Alu C 1x2x1x28:3 ↔ funnelFront:4
- Flush:1: Alu C Half Thick 1x3x1x20:1 ↔ plate:1
- Insert:298: Alu C Half Thick 1x3x1x20:2 ↔ plate:2
- Mate:98: Alu C 1x2x1x28:4 ↔ plate:2
- Insert:299: funnelFront:2 ↔ SScrew Star Smooth .375:44
- Insert:300: funnelFront:2 ↔ SScrew Star Smooth .375:42
- Insert:301: funnelFront:2 ↔ SScrew Star Smooth .375:40
- Insert:302: funnelFront:2 ↔ SScrew Star Smooth .375:41
- Insert:303: funnelFront:2 ↔ SScrew Star Smooth .375:43
- Insert:304: plate:1 ↔ SScrew Star Smooth .375:52
- Insert:305: plate:1 ↔ SScrew Star Smooth .375:53
- Insert:306: plate:1 ↔ SScrew Star Smooth .375:51
- Insert:307: plate:1 ↔ SScrew Star Smooth .375:49
- Insert:308: funnelFront:4 ↔ SScrew Star Smooth .375:50
- Insert:309: funnelFront:4 ↔ SScrew Star Smooth .375:47
- Insert:310: funnelFront:4 ↔ SScrew Star Smooth .375:45
- Insert:311: funnelFront:4 ↔ SScrew Star Smooth .375:46
- Insert:312: funnelFront:4 ↔ SScrew Star Smooth .375:48
- Insert:313: Alu C 1x2x1x26:1 ↔ SScrew Star Smooth 1.250:55
- Insert:314: Alu C 1x2x1x28:3 ↔ SScrew Star Smooth 1.250:54
- Insert:315: Alu C 1x2x1x26:1 ↔ Nut Nylock:16
- Insert:316: Alu C 1x2x1x28:3 ↔ Nut Nylock:17
- Insert:317: Alu C 1x2x1x26:2 ↔ SScrew Star Smooth 1.250:57
- Insert:318: Alu C 1x2x1x28:4 ↔ SScrew Star Smooth 1.250:56
- Insert:319: Alu C 1x2x1x26:2 ↔ Nut Nylock:18
- Insert:320: Alu C 1x2x1x28:4 ↔ Nut Nylock:19
- Insert:321: funnelFront:1 ↔ SScrew Star Smooth .375:58
- Insert:322: funnelFront:1 ↔ SScrew Star Smooth .375:60
- Insert:323: funnelFront:1 ↔ SScrew Star Smooth .375:62
- Insert:324: funnelFront:1 ↔ SScrew Star Smooth .375:61
- Insert:325: funnelFront:1 ↔ SScrew Star Smooth .375:59
- Insert:326: plate:2 ↔ SScrew Star Smooth .375:70
- Insert:327: plate:2 ↔ SScrew Star Smooth .375:71
- Insert:328: plate:2 ↔ SScrew Star Smooth .375:66
- Insert:329: plate:2 ↔ SScrew Star Smooth .375:64
- Insert:330: funnelFront:3 ↔ SScrew Star Smooth .375:65
- Insert:331: funnelFront:3 ↔ SScrew Star Smooth .375:69
- Insert:332: funnelFront:3 ↔ SScrew Star Smooth .375:68
- Insert:333: funnelFront:3 ↔ SScrew Star Smooth .375:63
- Insert:334: funnelFront:3 ↔ SScrew Star Smooth .375:67
## Named parameters: d164_d162 = 3.175 mm, d257_d254 = 0 mm, d258_d255 = 0 mm, d259_d254 = 0 mm, d260_d255 = 0 mm, d302_d300 = 0 mm, d473_d471 = 0 mm, d475_d471 = 0 mm, d477_d471 = 0 mm
